# Autodesk Inventor assembly: Fixture Assembly
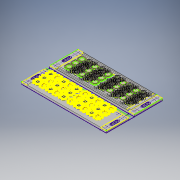
[picture p0: Inventor's stored thumbnail of the model, 180x180]
Saved by Autodesk Inventor 2016 (Build 200138000, 138)
## iProperties
Created: 2016-04-08
Part Number: Fixture Assembly
Document SubType Name: Assembly
Designer: Sam Clay
Author: Sam Clay
## Documents named in this file (6)
- Z:\enclosure\inventor\Fixture Assembly.iam
- Z:\enclosure\inventor\Fixture Base.ipt
- Z:\enclosure\inventor\Case Top.ipt
- Z:\enclosure\inventor\Case Bottom.ipt
- Z:\enclosure\inventor\Case Top Fixture.ipt
- Z:\enclosure\inventor\Case Bottom Fixture.ipt
## Components (61 placed, 5 different names)
1. Fixture Base:1 — Mate:12, Mate:13, Mate:15, Mate:16, Mate:18, Mate:26
2. Case Bottom:1 — Mate top pocket shell, Mate side pocket shell
3. Case Bottom:2
4. Case Bottom:3
5. Case Bottom:4
6. Case Bottom:5
7. Case Bottom:6
8. Case Top:2 — Mate side pocket shell, Mate top pocket shell, Mate:12, Mate:15
9. Case Top:3
10. Case Top:4
11. Case Top:5
12. Case Top:6
13. Case Top:7
14. Case Top:8 — Mate:17
15. Case Top:9
16. Case Top:10
17. Case Top Fixture:1 — Mate:9, Mate:25, Mate:26
18. Case Top Fixture:2
19. Case Top Fixture:3
20. Case Top Fixture:4
21. Case Top Fixture:5
22. Case Top Fixture:6
23. Case Top Fixture:7 — Mate:23, Mate:24
24. Case Top Fixture:8
25. Case Top Fixture:9
26. Case Bottom Fixture:1 — Mate:9, Mate:25
27. Case Bottom Fixture:2
28. Case Bottom Fixture:3
29. Case Bottom Fixture:4
30. Case Bottom Fixture:5
31. Case Bottom Fixture:6
32. Case Bottom:7 — Mate top pocket shell 2, Mate:13, Mate:16, Mate:17, Mate:19
33. Case Bottom:8
34. Case Bottom:9
35. Case Bottom:10
36. Case Bottom:11
37. Case Bottom:12
38. Case Bottom:13
39. Case Bottom:14
40. Case Bottom:15
41. Case Top:11 — Mate top pocket shell 2, Mate:18, Mate:19
42. Case Top:12
43. Case Top:13
44. Case Top:14
45. Case Top:15
46. Case Top:16
47. Case Bottom Fixture:7 — Mate:21, Mate:22, Mate:23, Mate:24
48. Case Bottom Fixture:8
49. Case Bottom Fixture:9
50. Case Bottom Fixture:10
51. Case Bottom Fixture:11
52. Case Bottom Fixture:12
53. Case Bottom Fixture:13
54. Case Bottom Fixture:14
55. Case Bottom Fixture:15
56. Case Top Fixture:10 — Mate:21, Mate:22
57. Case Top Fixture:11
58. Case Top Fixture:12
59. Case Top Fixture:13
60. Case Top Fixture:14
61. Case Top Fixture:15
## Component patterns: (6 elements, first: Case Bottom:1), (9 elements, first: Case Top:2), (9 elements, first: Case Top Fixture:1), (6 elements, first: Case Bottom Fixture:1), (9 elements, first: Case Bottom:7), (6 elements, first: Case Top:11), (9 elements, first: Case Bottom Fixture:7), (6 elements, first: Case Top Fixture:10)
## Relationships (17: Mate 17)
- Mate top pocket shell: Case Bottom:1 ↔ Case Top:2
- Mate top pocket shell 2: Case Bottom:7 ↔ Case Top:11
- Mate side pocket shell (6.604 mm): Case Bottom:1 ↔ Case Top:2
- Mate:9: Case Top Fixture:1 ↔ Case Bottom Fixture:1
- Mate:12: Fixture Base:1 ↔ Case Top:2
- Mate:13: Fixture Base:1 ↔ Case Bottom:7
- Mate:15 (3.175 mm): Fixture Base:1 ↔ Case Top:2
- Mate:16 (1.27 mm): Fixture Base:1 ↔ Case Bottom:7
- Mate:17 (25.4 mm): Case Top:8 ↔ Case Bottom:7
- Mate:19 (6.604 mm): Case Bottom:7 ↔ Case Top:11
- Mate:18: Fixture Base:1 ↔ Case Top:11
- Mate:21: Case Bottom Fixture:7 ↔ Case Top Fixture:10
- Mate:22 (6.604 mm): Case Bottom Fixture:7 ↔ Case Top Fixture:10
- Mate:23: Case Top Fixture:7 ↔ Case Bottom Fixture:7
- Mate:24 (25.4 mm): Case Top Fixture:7 ↔ Case Bottom Fixture:7
- Mate:25 (6.604 mm): Case Top Fixture:1 ↔ Case Bottom Fixture:1
- Mate:26 (16.51 mm): Fixture Base:1 ↔ Case Top Fixture:1
